# Autodesk Inventor assembly: Prototype1
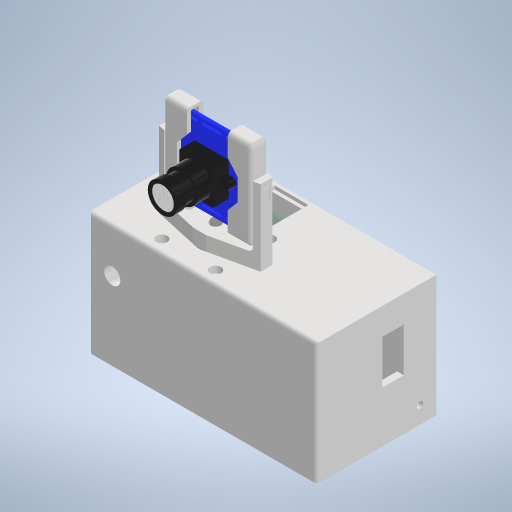
[picture p0: Inventor's stored thumbnail of the model, 512x512]
Saved by Autodesk Inventor 2023 (Build 270158000, 158)
## iProperties
Created: 2023-03-16
Part Number: Prototype1
Document SubType Name: Assembly
Designer: karpova
Author: karpova
## Documents named in this file (9)
- C:\_dev\24-transcription-study-assistant\cad-files\SeniorDesign_V0\Prototype1.iam
- C:\_dev\24-transcription-study-assistant\cad-files\SeniorDesign_V0\Board_Main.ipt
- C:\_dev\personal\BaseV1.ipt
- C:\_dev\personal\Enclosure_Base_v0.ipt
- C:\_dev\personal\Motor_Mount.ipt
- C:\_dev\personal\MotorMount_Standoff.ipt
- C:\_dev\24-transcription-study-assistant\cad-files\SeniorDesign_V0\StepperMotor.ipt
- C:\_dev\personal\Enclosure_Shell.ipt
- C:\_dev\24-transcription-study-assistant\cad-files\SeniorDesign_V0\TurretAssembly.iam
## Components (13 placed, 8 different names)
1. Board_Main:1 — Mate:1, Mate:2, Mate:3, Mate:4, Mate:5, Mate:6, Mate:7, Mate:8, Mate:9, Mate:10
2. BaseV1:1
3. Enclosure_Base_v0:1 — Mate:2, Mate:3, Flush:1, Mate:18, Mate:19, Mate:20
4. MotorMount_Standoff:2 — Mate:6, Mate:8
5. MotorMount_Standoff:3 — Mate:5, Mate:10
6. MotorMount_Standoff:4 — Mate:7, Mate:9, Mate:12, Mate:17
7. MotorMount_Standoff:5 — Mate:1, Mate:4, Mate:11
8. Motor_Mount:1 — Mate:11, Mate:12, Mate:17
9. StepperMotor:1
10. Enclosure_Shell:1 — Flush:1, Mate:21, Mate:22
11. Board_Main:2 — Mate:18, Mate:19, Mate:20
12. StepperMotor:2 — Mate:21
13. TurretAssembly:1 [sub-assembly] — Mate:22
## Relationships (19: Mate 18, Flush 1)
- Mate:1: Board_Main:1 ↔ MotorMount_Standoff:5
- Mate:2: Board_Main:1 ↔ Enclosure_Base_v0:1
- Mate:3: Board_Main:1 ↔ Enclosure_Base_v0:1
- Mate:4: Board_Main:1 ↔ MotorMount_Standoff:5
- Mate:5: Board_Main:1 ↔ MotorMount_Standoff:3
- Mate:6: Board_Main:1 ↔ MotorMount_Standoff:2
- Mate:7: Board_Main:1 ↔ MotorMount_Standoff:4
- Mate:8: Board_Main:1 ↔ MotorMount_Standoff:2
- Mate:9: Board_Main:1 ↔ MotorMount_Standoff:4
- Mate:10: Board_Main:1 ↔ MotorMount_Standoff:3
- Mate:11: MotorMount_Standoff:5 ↔ Motor_Mount:1
- Mate:12: MotorMount_Standoff:4 ↔ Motor_Mount:1
- Mate:17: MotorMount_Standoff:4 ↔ Motor_Mount:1
- Flush:1: Enclosure_Base_v0:1 ↔ Enclosure_Shell:1
- Mate:18: Enclosure_Base_v0:1 ↔ Board_Main:2
- Mate:19: Enclosure_Base_v0:1 ↔ Board_Main:2
- Mate:20: Enclosure_Base_v0:1 ↔ Board_Main:2
- Mate:21: Enclosure_Shell:1 ↔ StepperMotor:2
- Mate:22: Enclosure_Shell:1 ↔ TurretAssembly:1
## Named parameters: riserOffset = 3.175 mm
